# Autodesk Inventor assembly: CompleteRing
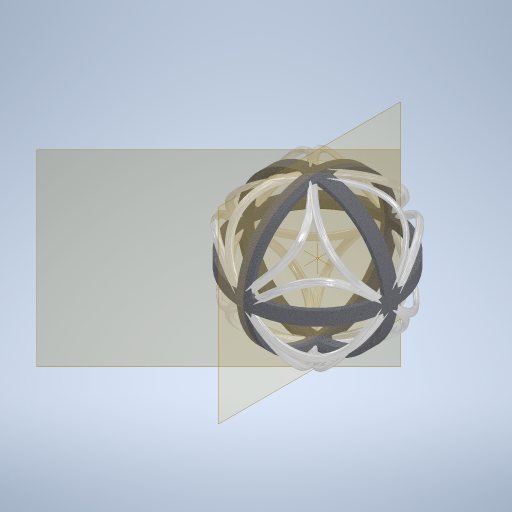
[picture p0: Inventor's stored thumbnail of the model, 512x512]
Saved by Autodesk Inventor 2023 (Build 270158000, 158)
## iProperties
Created: 2023-01-03
Part Number: CompleteRing
Document SubType Name: Assembly
Designer: redii
Author: redii
## Documents named in this file (8)
- C:\Users\redii\Desktop\CGM\My projectCube\OuterRing\CompleteRing.iam
- C:\Users\redii\Desktop\CGM\My projectCube\OuterRing\Ring.ipt
- C:\Users\redii\Desktop\CGM\My projectCube\OuterRing\RingSide.ipt
- C:\Users\redii\Desktop\CGM\My projectCube\OuterRing\RingSide_MIR.ipt
- C:\Users\redii\Desktop\CGM\My projectCube\OuterRing\RingSide_MIR1.ipt
- C:\Users\redii\Desktop\CGM\My projectCube\OuterRing\RingSide_MIR_MIR.ipt
- C:\Users\redii\Desktop\CGM\My projectCube\OuterRing\RingSide_MIR1_MIR.ipt
- C:\Users\redii\Desktop\CGM\My projectCube\OuterRing\RingSide_MIR_MIR_MIR.ipt
## Components (9 placed, 7 different names)
1. Ring:1 — Mate:7
2. Ring:2 — Mate:6
3. Ring:3
4. RingSide:1 — Mate:8, Mate:11
5. RingSide_MIR:1 — Mate:9, Mate:10
6. RingSide_MIR1:1 — Mate:14, Mate:15
7. RingSide_MIR_MIR:1 — Mate:16, Mate:17
8. RingSide_MIR1_MIR:1 — Mate:20, Mate:21
9. RingSide_MIR_MIR_MIR:1 — Mate:22, Mate:23
## Relationships (22: Mate 18, Angle 4)
- Mate:6: Ring:2
- Mate:7: Ring:1
- Mate:8: RingSide:1
- Mate:9: RingSide_MIR:1
- Mate:10: RingSide_MIR:1
- Mate:11: RingSide:1
- Mate:12
- Angle:1 (45 deg)
- Mate:13
- Angle:2 (45 deg)
- Mate:14: RingSide_MIR1:1
- Mate:15: RingSide_MIR1:1
- Mate:16: RingSide_MIR_MIR:1
- Mate:17: RingSide_MIR_MIR:1
- Mate:18
- Angle:3 (-45 deg)
- Mate:19
- Angle:4 (45 deg)
- Mate:20: RingSide_MIR1_MIR:1
- Mate:21: RingSide_MIR1_MIR:1
- Mate:22: RingSide_MIR_MIR_MIR:1
- Mate:23: RingSide_MIR_MIR_MIR:1
